# Autodesk Inventor assembly: Spinny disk assembly
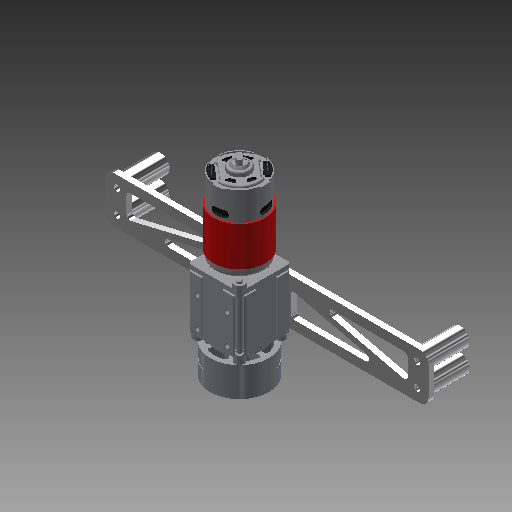
[picture p0: Inventor's stored thumbnail of the model, 512x512]
Saved by Autodesk Inventor 2019.4 (Build 234330000, 330)
## iProperties
Created: 2020-01-23
Part Number: Spinny disk assembly
Document SubType Name: Assembly
Designer: Mark
Mass: 264.042 g
Surface Area: 1766.54 cm^2
Volume: 264.042 cm^3
Density: 1 g/cm^3
Author: Mark
## Documents named in this file (6)
- C:\Users\Mark\Desktop\7738 Helion Engineering\7738-2020\Spinny disk assembly\Spinny disk assembly.iam
- C:\Users\Mark\Desktop\7738 Helion Engineering\7738-2020\Spinny disk assembly\2_OD_Straight_Flex_Wheel_217-6353.ipt
- C:\Users\Mark\Desktop\7738 Helion Engineering\7738-2020\Spinny disk assembly\2 Stage SD - 57 Sport.ipt
- C:\Users\Mark\Desktop\7738 Helion Engineering\7738-2020\Spinny disk assembly\am-3775a AndyMark RedLine Motor.ipt
- C:\Users\Mark\Desktop\7738 Helion Engineering\7738-2020\Spinny disk assembly\Back Plate Spinning thing.ipt
- C:\Users\Mark\Desktop\7738 Helion Engineering\7738-2020\Elevator MK2\Small Spacer.ipt
## Components (9 placed, 5 different names)
1. 2_OD_Straight_Flex_Wheel_217-6353:1 — Mate:1, Mate:2, Mate:3, Mate:4
2. 2 Stage SD - 57 Sport:1 — Mate:1, Mate:2, Mate:9, Mate:10, Mate:11, Mate:12, Mate:13
3. 2_OD_Straight_Flex_Wheel_217-6353:2 — Mate:3, Mate:4
4. am-3775a AndyMark RedLine Motor:1 — Mate:9, Mate:10
5. Back Plate Spinning thing:1 — Mate:11, Mate:12, Mate:13, Mate:14, Mate:15, Mate:16, Mate:17, Mate:18, Mate:19, Mate:20, Mate:21
6. Small Spacer:1 — Mate:14, Mate:15
7. Small Spacer:2 — Mate:16, Mate:17
8. Small Spacer:3 — Mate:20, Mate:21
9. Small Spacer:4 — Mate:18, Mate:19
## Relationships (17: Mate 17)
- Mate:1: 2_OD_Straight_Flex_Wheel_217-6353:1 ↔ 2 Stage SD - 57 Sport:1
- Mate:2 (1 mm): 2_OD_Straight_Flex_Wheel_217-6353:1 ↔ 2 Stage SD - 57 Sport:1
- Mate:3: 2_OD_Straight_Flex_Wheel_217-6353:1 ↔ 2_OD_Straight_Flex_Wheel_217-6353:2
- Mate:4: 2_OD_Straight_Flex_Wheel_217-6353:1 ↔ 2_OD_Straight_Flex_Wheel_217-6353:2
- Mate:9: 2 Stage SD - 57 Sport:1 ↔ am-3775a AndyMark RedLine Motor:1
- Mate:10: 2 Stage SD - 57 Sport:1 ↔ am-3775a AndyMark RedLine Motor:1
- Mate:11: 2 Stage SD - 57 Sport:1 ↔ Back Plate Spinning thing:1
- Mate:12: 2 Stage SD - 57 Sport:1 ↔ Back Plate Spinning thing:1
- Mate:13: 2 Stage SD - 57 Sport:1 ↔ Back Plate Spinning thing:1
- Mate:14: Back Plate Spinning thing:1 ↔ Small Spacer:1
- Mate:15: Back Plate Spinning thing:1 ↔ Small Spacer:1
- Mate:16: Back Plate Spinning thing:1 ↔ Small Spacer:2
- Mate:17: Back Plate Spinning thing:1 ↔ Small Spacer:2
- Mate:18: Back Plate Spinning thing:1 ↔ Small Spacer:4
- Mate:19: Back Plate Spinning thing:1 ↔ Small Spacer:4
- Mate:20: Back Plate Spinning thing:1 ↔ Small Spacer:3
- Mate:21: Back Plate Spinning thing:1 ↔ Small Spacer:3
